# Autodesk Inventor assembly: face
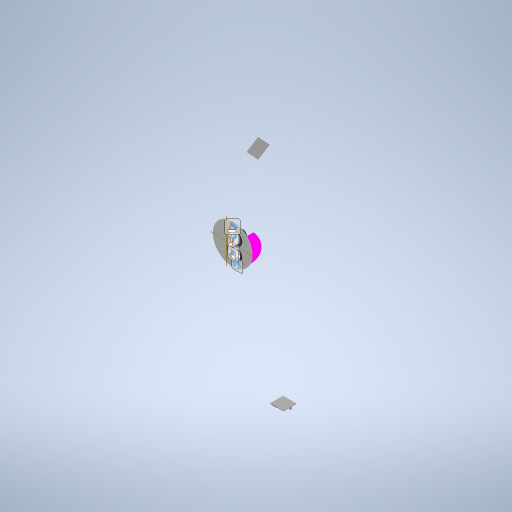
[picture p0: Inventor's stored thumbnail of the model, 512x512]
Saved by Autodesk Inventor 2023.2 (Build 272271030, 271C)
## iProperties
Created: 2024-01-26
Part Number: face
Document SubType Name: Assembly
Designer: I9232
Author: I9232
## Documents named in this file (15)
- D:\!project\fox_n_crow_construction\crow\face\face.iam
- D:\!project\fox_n_crow_construction\crow\face\Сборка глаза вороны.iam
- D:\!project\fox_n_crow_construction\crow\face\Деталь1.ipt
- D:\!project\fox_n_crow_construction\crow\face\Платформа для крыльев лево.ipt
- D:\!project\fox_n_crow_construction\crow\face\Платформа для крыльев право.ipt
- D:\!project\fox_n_crow_construction\crow\face\Сыр.ipt
- D:\!project\fox_n_crow_construction\crow\face\Веер.ipt
- D:\!project\fox_n_crow_construction\crow\face\боковые стороны головы.ipt
- D:\!project\fox_n_crow_construction\crow\face\servoDS3115mg.iam
- D:\!project\fox_n_crow_construction\crow\face\SERVO ARM HORN 25T ALUMINIUM\SERVO ARM HORN 25T ALUMINIUM.ipt
- D:\!project\fox_n_crow_construction\crow\face\Крепление рычага к лицу.ipt
- D:\!project\fox_n_crow_construction\crow\face\Рычаг.ipt
- D:\!project\fox_n_crow_construction\crow\face\Лицо низ.ipt
- D:\!project\fox_n_crow_construction\crow\face\Лицо верх.ipt
- D:\!project\fox_n_crow_construction\crow\face\door_hinge.iam
## Components (15 placed, 14 different names)
1. Сборка глаза вороны:1 [sub-assembly] — Заподлицо:1, Совмещение:5
2. Платформа глаз — Заподлицо:1, Совмещение:4, Совмещение:5, Заподлицо:4, Заподлицо:5, Заподлицо:6
3. Платформа для крыльев лево:1
4. Платформа для крыльев право:1 — Жесткий:1
5. Сыр:1
6. Веер:1 — Жесткий:1
7. Веер:2
8. боковые стороны головы:1 — Совмещение:4, Совмещение:6, Совмещение:7, Совмещение:8
9. servoDS3115mg:1 [sub-assembly] — Совмещение:6, Совмещение:7, Совмещение:8, Совмещение:15, Совмещение:16
10. SERVO ARM HORN 25T ALUMINIUM:1 — Совмещение:15, Цилиндрический:4, Совмещение:16, Совмещение:17
11. Крепление рычага к лицу:1 — Совмещение:12, Заподлицо:7, Совмещение:14, Цилиндрический:3
12. Рычаг:1 — Цилиндрический:3, Цилиндрический:4, Совмещение:17
13. Лицо низ:1 — Цилиндрический:2, Угол:2, Совмещение:12, Заподлицо:7, Совмещение:13, Совмещение:14
14. Лицо верх:1 — Заподлицо:4, Заподлицо:5, Заподлицо:6, Совмещение:10, Цилиндрический:1, Угол:1, Угол:2
15. door_hinge:1 [sub-assembly] — Совмещение:10, Цилиндрический:1, Угол:1, Цилиндрический:2, Совмещение:13
## Relationships (24: Mate 12, Flush 5, CylindricalJoint 4, Angle 2, WeldJoint 1)
- Заподлицо:1 [Flush]: Сборка глаза вороны:1 ↔ Платформа глаз
- Жесткий:1 [WeldJoint]: Платформа для крыльев право:1 ↔ Веер:1
- Совмещение:4 [Mate]: Платформа глаз ↔ боковые стороны головы:1
- Совмещение:5 [Mate]: Сборка глаза вороны:1 ↔ Платформа глаз
- Совмещение:6 [Mate]: боковые стороны головы:1 ↔ servoDS3115mg:1
- Совмещение:7 [Mate]: боковые стороны головы:1 ↔ servoDS3115mg:1
- Совмещение:8 [Mate]: боковые стороны головы:1 ↔ servoDS3115mg:1
- Заподлицо:4 [Flush]: Платформа глаз ↔ Лицо верх:1
- Заподлицо:5 [Flush]: Платформа глаз ↔ Лицо верх:1
- Заподлицо:6 [Flush]: Платформа глаз ↔ Лицо верх:1
- Совмещение:10 [Mate]: Лицо верх:1 ↔ door_hinge:1
- Цилиндрический:1 [CylindricalJoint]: Лицо верх:1 ↔ door_hinge:1
- Угол:1 [Angle] (180 deg): Лицо верх:1 ↔ door_hinge:1
- Цилиндрический:2 [CylindricalJoint]: Лицо низ:1 ↔ door_hinge:1
- Угол:2 [Angle] (0 deg): Лицо низ:1 ↔ Лицо верх:1
- Совмещение:12 [Mate]: Крепление рычага к лицу:1 ↔ Лицо низ:1
- Заподлицо:7 [Flush]: Крепление рычага к лицу:1 ↔ Лицо низ:1
- Совмещение:13 [Mate]: Лицо низ:1 ↔ door_hinge:1
- Совмещение:14 [Mate]: Крепление рычага к лицу:1 ↔ Лицо низ:1
- Цилиндрический:3 [CylindricalJoint]: Крепление рычага к лицу:1 ↔ Рычаг:1
- Совмещение:15 [Mate]: servoDS3115mg:1 ↔ SERVO ARM HORN 25T ALUMINIUM:1
- Цилиндрический:4 [CylindricalJoint]: SERVO ARM HORN 25T ALUMINIUM:1 ↔ Рычаг:1
- Совмещение:16 [Mate]: servoDS3115mg:1 ↔ SERVO ARM HORN 25T ALUMINIUM:1
- Совмещение:17 [Mate]: SERVO ARM HORN 25T ALUMINIUM:1 ↔ Рычаг:1
